# Autodesk Inventor assembly: 556814 EGC-80-700-TB-KF-0H-GK_(0)
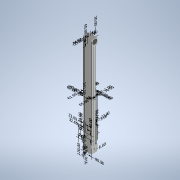
[picture p0: Inventor's stored thumbnail of the model, 180x180]
Saved by Autodesk Inventor 2021 (Build 250183000, 183)
## iProperties
Category: PARTsolutions
Company: FESTO
Created: 2026-04-25
Part Number: 556814 EGC-80-700-TB-KF-0H-GK_(0)
Catalog Web Link: www.3dfindit.com
Description: EGC-TB (m)-Toothed belt axis, Modular system
Vendor: FESTO
Document SubType Name: Assembly
Designer: psAdmin
Manufacturer: FESTO
Mass: 7340 g
Surface Area: 4784.22 cm^2
Volume: 4077.02 cm^3
Density: 1.80034 g/cm^3
Title: 556814 EGC-80-700-TB-KF-0H-GK
Author: Cadenas PARTsolutions
Comments: Toothed belt axis, Modular system
PSOL_IDENT_0: {ATYP=ASSISTANT},{DATA=script=$CADENAS_DATA/23d-libs/festo/webfesto.vbb&M_FAMILY=EGC&M_GROUP=01&M_PA
PSOL_IDENT_1: RTNO=556814&IDCODE1=EGC-80-700-TB-KF-0H-GK&IDCODE2=&HUB=700&N_EGC_TB_HR=0&C_EGC_TB_HEAD=EGC&C_EGC_TB
PSOL_IDENT_2: _BG=80&C_EGC_TB_FKT=TB&C_EGC_TB_FHR=KF&CH_EGC_HR=0H&C_EGC_TB_SL=GK&customer_number_cns=&MATES=1&LOD=
PSOL_IDENT_3: HI&LOCKERP=0}
NB: 556814 EGC-80-700-TB-KF-0H-GK_(0)
NN: EGC-TB (m)
NT: Toothed belt axis, Modular system
NBSYN: $TNR. $TYP1._($HUBST.)
LINA: 556814 EGC-80-700-TB-KF-0H-GK
CATALOG: Festo
TNR: 556814
TYP: EGC-80
HUB: 700
HUBST: 0
FKT: TB
FHR: KF
HRTB: 0
SL: GK
ZSL: -
ZSR: -
SA: -
WMS: -
FSA: -
BEA: -
AZM: -
ATEX: -
B1: 82
B2: 72.6
B3: 22
B4: 40
B5: 60
B9: 1
B11: 32.5
B12: 24.5
B13: 3
B14: 98.4
B15: 64.4
B16: 17.4
B17: 39.4
B18: 25
B19: 46
D1: 48
D2: 16
D3: 46.5
D4: 25
D5: 9
D6: M5
D7: M5
D8: 5
D9: M6
D10: M3
H1: 76.5
H2: 34.5
H3: 65
H4: 61.5
H5: 17.5
H6: 15
H7: 35
H11: 48
H12: 24.4
H13: 15
H14: 5
H15: 87.5
H16: 11
H17: 39.6
L1: 986
L2: 143
L3: 65
L4: 46
L5: 30
L6: 2
L8: 3
L9: 13
L11: 86
L12: 72
L13: 47
L14: 45
L15: 30
L17: 63
T1: 2.1
T2: 27
T3: 31.25
T4: 4
T5: 32
T6: 2.1
T7: 10
T8: 10
T9: 3.1
CNSMASSEXACT: 7.34
SUPPLIER: FESTO
ARTICLENO: 556814 EGC-80-700-TB-KF-0H-GK_(0)
BOMINFO: 556814 EGC-80-700-TB-KF-0H-GK
CREATOR: CADENAS GmbH
## Documents named in this file (7)
- e:\temp\worker_COMMON_205\temp\tmp_5268_18_mTt2z\format_0\556814 EGC-80-700-TB-KF-0H-GK_(0).iam
- e:\temp\worker_COMMON_205\temp\tmp_5268_18_mTt2z\format_0\EGC-80-TB85678GK0--0---0_0_R0L22000.ipt
- e:\temp\worker_COMMON_205\temp\tmp_5268_18_mTt2z\format_0\EGC-80-TB-KF___(0_0_0_Deckel LI).ipt
- e:\temp\worker_COMMON_205\temp\tmp_5268_18_mTt2z\format_0\EGC-80-TB-KF_(AK).ipt
- e:\temp\worker_COMMON_205\temp\tmp_5268_18_mTt2z\format_0\EGC-80-TB-KF__(CUP).ipt
- e:\temp\worker_COMMON_205\temp\tmp_5268_18_mTt2z\format_0\EGC-80-TB-KF___(0_0_Deckel RE).ipt
- e:\temp\worker_COMMON_205\temp\tmp_5268_18_mTt2z\format_0\EGC-80-GK-GPTB1--------(0).ipt
## Components (9 placed, 6 different names)
1. EGC-80-TB85678GK0--0---0_0_R0L22000:1 — ZR1_XY@1 <-> DL_XY@2, ZR1_Z@1 <-> DL_Z@2, ZR1_YZ@1 <-> DL_YZ@2, ZR2_XY@1 <-> DR_XY@6, ZR2_Z@1 <-> DR_Z@6, ZR2_YZ@1 <-> DR_YZ@6, TO_SLIDE_XY@1 <-> SCHLITTEN_XY@9, TO_SLIDE_Z@1 <-> SCHLITTEN_Z@9, TO_SLIDE_YZ@1 <-> SCHLITTEN_YZ@9
2. EGC-80-TB-KF___(0_0_0_Deckel LI):1 — ZR1_XY@1 <-> DL_XY@2, ZR1_Z@1 <-> DL_Z@2, ZR1_YZ@1 <-> DL_YZ@2, TO_AK_XY@2 <-> AK_XY@3, TO_AK_Z@2 <-> AK_Z@3, TO_AK_YZ@2 <-> AK_YZ@3, CUP1_XY@2 <-> CUP_XY@4, CUP1_Z@2 <-> CUP_Z@4, CUP1_YZ@2 <-> CUP_YZ@4, CUP2_XY@2 <-> CUP_XY@5, CUP2_Z@2 <-> CUP_Z@5, CUP2_YZ@2 <-> CUP_YZ@5
3. EGC-80-TB-KF_(AK):1 — TO_AK_XY@2 <-> AK_XY@3, TO_AK_Z@2 <-> AK_Z@3, TO_AK_YZ@2 <-> AK_YZ@3
4. EGC-80-TB-KF__(CUP):1 — CUP1_XY@2 <-> CUP_XY@4, CUP1_Z@2 <-> CUP_Z@4, CUP1_YZ@2 <-> CUP_YZ@4
5. EGC-80-TB-KF__(CUP):2 — CUP2_XY@2 <-> CUP_XY@5, CUP2_Z@2 <-> CUP_Z@5, CUP2_YZ@2 <-> CUP_YZ@5
6. EGC-80-TB-KF___(0_0_Deckel RE):1 — ZR2_XY@1 <-> DR_XY@6, ZR2_Z@1 <-> DR_Z@6, ZR2_YZ@1 <-> DR_YZ@6, TO_AK_XY@6 <-> AK_XY@7, TO_AK_Z@6 <-> AK_Z@7, TO_AK_YZ@6 <-> AK_YZ@7, CUP1_XY@6 <-> CUP_XY@8, CUP1_Z@6 <-> CUP_Z@8, CUP1_YZ@6 <-> CUP_YZ@8
7. EGC-80-TB-KF_(AK):2 — TO_AK_XY@6 <-> AK_XY@7, TO_AK_Z@6 <-> AK_Z@7, TO_AK_YZ@6 <-> AK_YZ@7
8. EGC-80-TB-KF__(CUP):3 — CUP1_XY@6 <-> CUP_XY@8, CUP1_Z@6 <-> CUP_Z@8, CUP1_YZ@6 <-> CUP_YZ@8
9. EGC-80-GK-GPTB1--------(0):1 — TO_SLIDE_XY@1 <-> SCHLITTEN_XY@9, TO_SLIDE_Z@1 <-> SCHLITTEN_Z@9, TO_SLIDE_YZ@1 <-> SCHLITTEN_YZ@9
## Relationships (24: Mate 13, Angle 8, Flush 3)
- ZR1_XY@1 <-> DL_XY@2 [Mate]: EGC-80-TB85678GK0--0---0_0_R0L22000:1 ↔ EGC-80-TB-KF___(0_0_0_Deckel LI):1
- ZR1_Z@1 <-> DL_Z@2 [Mate]: EGC-80-TB85678GK0--0---0_0_R0L22000:1 ↔ EGC-80-TB-KF___(0_0_0_Deckel LI):1
- ZR1_YZ@1 <-> DL_YZ@2 [Angle] (0 deg): EGC-80-TB85678GK0--0---0_0_R0L22000:1 ↔ EGC-80-TB-KF___(0_0_0_Deckel LI):1
- TO_AK_XY@2 <-> AK_XY@3 [Mate]: EGC-80-TB-KF___(0_0_0_Deckel LI):1 ↔ EGC-80-TB-KF_(AK):1
- TO_AK_Z@2 <-> AK_Z@3 [Mate]: EGC-80-TB-KF___(0_0_0_Deckel LI):1 ↔ EGC-80-TB-KF_(AK):1
- TO_AK_YZ@2 <-> AK_YZ@3 [Angle] (0 deg): EGC-80-TB-KF___(0_0_0_Deckel LI):1 ↔ EGC-80-TB-KF_(AK):1
- CUP1_XY@2 <-> CUP_XY@4 [Flush]: EGC-80-TB-KF___(0_0_0_Deckel LI):1 ↔ EGC-80-TB-KF__(CUP):1
- CUP1_Z@2 <-> CUP_Z@4 [Mate]: EGC-80-TB-KF___(0_0_0_Deckel LI):1 ↔ EGC-80-TB-KF__(CUP):1
- CUP1_YZ@2 <-> CUP_YZ@4 [Angle] (0 deg): EGC-80-TB-KF___(0_0_0_Deckel LI):1 ↔ EGC-80-TB-KF__(CUP):1
- CUP2_XY@2 <-> CUP_XY@5 [Flush]: EGC-80-TB-KF___(0_0_0_Deckel LI):1 ↔ EGC-80-TB-KF__(CUP):2
- CUP2_Z@2 <-> CUP_Z@5 [Mate]: EGC-80-TB-KF___(0_0_0_Deckel LI):1 ↔ EGC-80-TB-KF__(CUP):2
- CUP2_YZ@2 <-> CUP_YZ@5 [Angle] (0 deg): EGC-80-TB-KF___(0_0_0_Deckel LI):1 ↔ EGC-80-TB-KF__(CUP):2
- ZR2_XY@1 <-> DR_XY@6 [Mate]: EGC-80-TB85678GK0--0---0_0_R0L22000:1 ↔ EGC-80-TB-KF___(0_0_Deckel RE):1
- ZR2_Z@1 <-> DR_Z@6 [Mate]: EGC-80-TB85678GK0--0---0_0_R0L22000:1 ↔ EGC-80-TB-KF___(0_0_Deckel RE):1
- ZR2_YZ@1 <-> DR_YZ@6 [Angle] (0 deg): EGC-80-TB85678GK0--0---0_0_R0L22000:1 ↔ EGC-80-TB-KF___(0_0_Deckel RE):1
- TO_AK_XY@6 <-> AK_XY@7 [Mate]: EGC-80-TB-KF___(0_0_Deckel RE):1 ↔ EGC-80-TB-KF_(AK):2
- TO_AK_Z@6 <-> AK_Z@7 [Mate]: EGC-80-TB-KF___(0_0_Deckel RE):1 ↔ EGC-80-TB-KF_(AK):2
- TO_AK_YZ@6 <-> AK_YZ@7 [Angle] (0 deg): EGC-80-TB-KF___(0_0_Deckel RE):1 ↔ EGC-80-TB-KF_(AK):2
- CUP1_XY@6 <-> CUP_XY@8 [Flush]: EGC-80-TB-KF___(0_0_Deckel RE):1 ↔ EGC-80-TB-KF__(CUP):3
- CUP1_Z@6 <-> CUP_Z@8 [Mate]: EGC-80-TB-KF___(0_0_Deckel RE):1 ↔ EGC-80-TB-KF__(CUP):3
- CUP1_YZ@6 <-> CUP_YZ@8 [Angle] (0 deg): EGC-80-TB-KF___(0_0_Deckel RE):1 ↔ EGC-80-TB-KF__(CUP):3
- TO_SLIDE_XY@1 <-> SCHLITTEN_XY@9 [Mate]: EGC-80-TB85678GK0--0---0_0_R0L22000:1 ↔ EGC-80-GK-GPTB1--------(0):1
- TO_SLIDE_Z@1 <-> SCHLITTEN_Z@9 [Mate]: EGC-80-TB85678GK0--0---0_0_R0L22000:1 ↔ EGC-80-GK-GPTB1--------(0):1
- TO_SLIDE_YZ@1 <-> SCHLITTEN_YZ@9 [Angle] (0 deg): EGC-80-TB85678GK0--0---0_0_R0L22000:1 ↔ EGC-80-GK-GPTB1--------(0):1
